# Autodesk Inventor assembly: Raspberry Pi 3
(part 2 of 2)
- C:\Users\jferner\Downloads\raspberry-pi-3-model-b-reference-design-solidworks-cad-rpi-raspberrypi-raspberry-pi-1.snapshot.83\Solidworks Complete Assembly\Raspberry Pi 3320.ipt
- C:\Users\jferner\Downloads\raspberry-pi-3-model-b-reference-design-solidworks-cad-rpi-raspberrypi-raspberry-pi-1.snapshot.83\Solidworks Complete Assembly\Raspberry Pi 3321.ipt
- C:\Users\jferner\Downloads\raspberry-pi-3-model-b-reference-design-solidworks-cad-rpi-raspberrypi-raspberry-pi-1.snapshot.83\Solidworks Complete Assembly\Raspberry Pi 3322.ipt
- C:\Users\jferner\Downloads\raspberry-pi-3-model-b-reference-design-solidworks-cad-rpi-raspberrypi-raspberry-pi-1.snapshot.83\Solidworks Complete Assembly\Raspberry Pi 3323.ipt
- C:\Users\jferner\Downloads\raspberry-pi-3-model-b-reference-design-solidworks-cad-rpi-raspberrypi-raspberry-pi-1.snapshot.83\Solidworks Complete Assembly\Raspberry Pi 3324.ipt
- C:\Users\jferner\Downloads\raspberry-pi-3-model-b-reference-design-solidworks-cad-rpi-raspberrypi-raspberry-pi-1.snapshot.83\Solidworks Complete Assembly\Raspberry Pi 3325.ipt
- C:\Users\jferner\Downloads\raspberry-pi-3-model-b-reference-design-solidworks-cad-rpi-raspberrypi-raspberry-pi-1.snapshot.83\Solidworks Complete Assembly\Raspberry Pi 3326.ipt
- C:\Users\jferner\Downloads\raspberry-pi-3-model-b-reference-design-solidworks-cad-rpi-raspberrypi-raspberry-pi-1.snapshot.83\Solidworks Complete Assembly\Raspberry Pi 3327.ipt
- C:\Users\jferner\Downloads\raspberry-pi-3-model-b-reference-design-solidworks-cad-rpi-raspberrypi-raspberry-pi-1.snapshot.83\Solidworks Complete Assembly\Raspberry Pi 3328.ipt
- C:\Users\jferner\Downloads\raspberry-pi-3-model-b-reference-design-solidworks-cad-rpi-raspberrypi-raspberry-pi-1.snapshot.83\Solidworks Complete Assembly\Raspberry Pi 3329.ipt
- C:\Users\jferner\Downloads\raspberry-pi-3-model-b-reference-design-solidworks-cad-rpi-raspberrypi-raspberry-pi-1.snapshot.83\Solidworks Complete Assembly\Raspberry Pi 3330.ipt
- C:\Users\jferner\Downloads\raspberry-pi-3-model-b-reference-design-solidworks-cad-rpi-raspberrypi-raspberry-pi-1.snapshot.83\Solidworks Complete Assembly\Raspberry Pi 3331.ipt
- C:\Users\jferner\Downloads\raspberry-pi-3-model-b-reference-design-solidworks-cad-rpi-raspberrypi-raspberry-pi-1.snapshot.83\Solidworks Complete Assembly\Raspberry Pi 3332.ipt
- C:\Users\jferner\Downloads\raspberry-pi-3-model-b-reference-design-solidworks-cad-rpi-raspberrypi-raspberry-pi-1.snapshot.83\Solidworks Complete Assembly\Raspberry Pi 3333.ipt
- C:\Users\jferner\Downloads\raspberry-pi-3-model-b-reference-design-solidworks-cad-rpi-raspberrypi-raspberry-pi-1.snapshot.83\Solidworks Complete Assembly\Raspberry Pi 3334.ipt
- C:\Users\jferner\Downloads\raspberry-pi-3-model-b-reference-design-solidworks-cad-rpi-raspberrypi-raspberry-pi-1.snapshot.83\Solidworks Complete Assembly\Raspberry Pi 3335.ipt
- C:\Users\jferner\Downloads\raspberry-pi-3-model-b-reference-design-solidworks-cad-rpi-raspberrypi-raspberry-pi-1.snapshot.83\Solidworks Complete Assembly\Raspberry Pi 3336.ipt
- C:\Users\jferner\Downloads\raspberry-pi-3-model-b-reference-design-solidworks-cad-rpi-raspberrypi-raspberry-pi-1.snapshot.83\Solidworks Complete Assembly\Raspberry Pi 3337.ipt
- C:\Users\jferner\Downloads\raspberry-pi-3-model-b-reference-design-solidworks-cad-rpi-raspberrypi-raspberry-pi-1.snapshot.83\Solidworks Complete Assembly\Raspberry Pi 3338.ipt
- C:\Users\jferner\Downloads\raspberry-pi-3-model-b-reference-design-solidworks-cad-rpi-raspberrypi-raspberry-pi-1.snapshot.83\Solidworks Complete Assembly\Raspberry Pi 3339.ipt
- C:\Users\jferner\Downloads\raspberry-pi-3-model-b-reference-design-solidworks-cad-rpi-raspberrypi-raspberry-pi-1.snapshot.83\Solidworks Complete Assembly\Raspberry Pi 3340.ipt
- C:\Users\jferner\Downloads\raspberry-pi-3-model-b-reference-design-solidworks-cad-rpi-raspberrypi-raspberry-pi-1.snapshot.83\Solidworks Complete Assembly\Raspberry Pi 3341.ipt
- C:\Users\jferner\Downloads\raspberry-pi-3-model-b-reference-design-solidworks-cad-rpi-raspberrypi-raspberry-pi-1.snapshot.83\Solidworks Complete Assembly\Raspberry Pi 3342.ipt
- C:\Users\jferner\Downloads\raspberry-pi-3-model-b-reference-design-solidworks-cad-rpi-raspberrypi-raspberry-pi-1.snapshot.83\Solidworks Complete Assembly\Raspberry Pi 3343.ipt
- C:\Users\jferner\Downloads\raspberry-pi-3-model-b-reference-design-solidworks-cad-rpi-raspberrypi-raspberry-pi-1.snapshot.83\Solidworks Complete Assembly\Raspberry Pi 3344.ipt
- C:\Users\jferner\Downloads\raspberry-pi-3-model-b-reference-design-solidworks-cad-rpi-raspberrypi-raspberry-pi-1.snapshot.83\Solidworks Complete Assembly\Raspberry Pi 3345.ipt
- C:\Users\jferner\Downloads\raspberry-pi-3-model-b-reference-design-solidworks-cad-rpi-raspberrypi-raspberry-pi-1.snapshot.83\Solidworks Complete Assembly\Raspberry Pi 3346.ipt
- C:\Users\jferner\Downloads\raspberry-pi-3-model-b-reference-design-solidworks-cad-rpi-raspberrypi-raspberry-pi-1.snapshot.83\Solidworks Complete Assembly\Raspberry Pi 3347.ipt
- C:\Users\jferner\Downloads\raspberry-pi-3-model-b-reference-design-solidworks-cad-rpi-raspberrypi-raspberry-pi-1.snapshot.83\Solidworks Complete Assembly\Raspberry Pi 3348.ipt
- C:\Users\jferner\Downloads\raspberry-pi-3-model-b-reference-design-solidworks-cad-rpi-raspberrypi-raspberry-pi-1.snapshot.83\Solidworks Complete Assembly\Raspberry Pi 3349.ipt
- C:\Users\jferner\Downloads\raspberry-pi-3-model-b-reference-design-solidworks-cad-rpi-raspberrypi-raspberry-pi-1.snapshot.83\Solidworks Complete Assembly\Raspberry Pi 3350.ipt
- C:\Users\jferner\Downloads\raspberry-pi-3-model-b-reference-design-solidworks-cad-rpi-raspberrypi-raspberry-pi-1.snapshot.83\Solidworks Complete Assembly\Raspberry Pi 3351.ipt
- C:\Users\jferner\Downloads\raspberry-pi-3-model-b-reference-design-solidworks-cad-rpi-raspberrypi-raspberry-pi-1.snapshot.83\Solidworks Complete Assembly\Raspberry Pi 3352.ipt
- C:\Users\jferner\Downloads\raspberry-pi-3-model-b-reference-design-solidworks-cad-rpi-raspberrypi-raspberry-pi-1.snapshot.83\Solidworks Complete Assembly\Raspberry Pi 3353.ipt
- C:\Users\jferner\Downloads\raspberry-pi-3-model-b-reference-design-solidworks-cad-rpi-raspberrypi-raspberry-pi-1.snapshot.83\Solidworks Complete Assembly\Raspberry Pi 3354.ipt
- C:\Users\jferner\Downloads\raspberry-pi-3-model-b-reference-design-solidworks-cad-rpi-raspberrypi-raspberry-pi-1.snapshot.83\Solidworks Complete Assembly\Raspberry Pi 3357.ipt
- C:\Users\jferner\Downloads\raspberry-pi-3-model-b-reference-design-solidworks-cad-rpi-raspberrypi-raspberry-pi-1.snapshot.83\Solidworks Complete Assembly\Raspberry Pi 3355.ipt
- C:\Users\jferner\Downloads\raspberry-pi-3-model-b-reference-design-solidworks-cad-rpi-raspberrypi-raspberry-pi-1.snapshot.83\Solidworks Complete Assembly\Raspberry Pi 3356.ipt
- C:\Users\jferner\Downloads\raspberry-pi-3-model-b-reference-design-solidworks-cad-rpi-raspberrypi-raspberry-pi-1.snapshot.83\Solidworks Complete Assembly\Part2^Raspberry Pi 3.ipt
- C:\Users\jferner\Downloads\raspberry-pi-3-model-b-reference-design-solidworks-cad-rpi-raspberrypi-raspberry-pi-1.snapshot.83\Solidworks Complete Assembly\Raspberry Pi 3360.ipt
- C:\Users\jferner\Downloads\raspberry-pi-3-model-b-reference-design-solidworks-cad-rpi-raspberrypi-raspberry-pi-1.snapshot.83\Solidworks Complete Assembly\Part4^Raspberry Pi 3.ipt
- C:\Users\jferner\Downloads\raspberry-pi-3-model-b-reference-design-solidworks-cad-rpi-raspberrypi-raspberry-pi-1.snapshot.83\Solidworks Complete Assembly\Solder2.ipt
- C:\Users\jferner\Downloads\raspberry-pi-3-model-b-reference-design-solidworks-cad-rpi-raspberrypi-raspberry-pi-1.snapshot.83\Solidworks Complete Assembly\Raspberry Pi 3358.ipt
- C:\Users\jferner\Downloads\raspberry-pi-3-model-b-reference-design-solidworks-cad-rpi-raspberrypi-raspberry-pi-1.snapshot.83\Solidworks Complete Assembly\Raspberry Pi 3359.ipt
- C:\Users\jferner\Downloads\raspberry-pi-3-model-b-reference-design-solidworks-cad-rpi-raspberrypi-raspberry-pi-1.snapshot.83\Solidworks Complete Assembly\mf-msmf050-2.ipt
- C:\Users\jferner\Downloads\raspberry-pi-3-model-b-reference-design-solidworks-cad-rpi-raspberrypi-raspberry-pi-1.snapshot.83\Solidworks Complete Assembly\Raspberry Pi 3163_smaller.ipt
- C:\Users\jferner\Downloads\raspberry-pi-3-model-b-reference-design-solidworks-cad-rpi-raspberrypi-raspberry-pi-1.snapshot.83\Solidworks Complete Assembly\Raspberry Pi 353_smaller.ipt
- C:\Users\jferner\Downloads\raspberry-pi-3-model-b-reference-design-solidworks-cad-rpi-raspberrypi-raspberry-pi-1.snapshot.83\Solidworks Complete Assembly\Raspberry Pi 3164_small.ipt
- C:\Users\jferner\Downloads\raspberry-pi-3-model-b-reference-design-solidworks-cad-rpi-raspberrypi-raspberry-pi-1.snapshot.83\Solidworks Complete Assembly\Raspberry Pi 3165_smaller.ipt
- C:\Users\jferner\Downloads\raspberry-pi-3-model-b-reference-design-solidworks-cad-rpi-raspberrypi-raspberry-pi-1.snapshot.83\Solidworks Complete Assembly\Raspberry Pi 3141_smaller.ipt
- C:\Users\jferner\Downloads\raspberry-pi-3-model-b-reference-design-solidworks-cad-rpi-raspberrypi-raspberry-pi-1.snapshot.83\Solidworks Complete Assembly\Assem1^Raspberry Pi 3.iam
- C:\Users\jferner\Downloads\raspberry-pi-3-model-b-reference-design-solidworks-cad-rpi-raspberrypi-raspberry-pi-1.snapshot.83\Solidworks Complete Assembly\raspberry_pi_B+_(microsd2).ipt
## Components (634 placed, 323 different names)
1. Raspberry Pi 3157:1
2. Raspberry Pi 3242:1
3. Raspberry Pi 3266:1
4. raspberry_pi_3(bar_180_2x20):2
5. RPi3_ModelB v1:1 [sub-assembly]
6. Raspberry Pi 312:1
7. Raspberry Pi 314:1
8. Raspberry Pi 3172:1
9. Raspberry Pi 3173:1
10. Raspberry Pi 3174:1
11. Raspberry Pi 3175:1
12. Raspberry Pi 3176:1
13. Raspberry Pi 3177:1
14. Raspberry Pi 3178:1
15. Raspberry Pi 3179:1
16. Raspberry Pi 3180:1
17. Raspberry Pi 3181:1
18. Raspberry Pi 3182:1
19. Raspberry Pi 3183:1
20. Raspberry Pi 3184:1
21. Raspberry Pi 3185:1
22. Raspberry Pi 3186:1
23. Raspberry Pi 3187:1
24. Raspberry Pi 3188:1
25. Raspberry Pi 3189:1
26. Raspberry Pi 3190:1
27. Raspberry Pi 3191:1
28. Raspberry Pi 3192:1
29. Raspberry Pi 3193:1
30. Raspberry Pi 3194:1
31. Raspberry Pi 3195:1
32. Raspberry Pi 3196:1
33. Raspberry Pi 3197:1
34. Raspberry Pi 3198:1
35. Raspberry Pi 3199:1
36. Raspberry Pi 3200:1
37. Raspberry Pi 3201:1
38. Raspberry Pi 3202:1
39. Raspberry Pi 3203:1
40. Raspberry Pi 3204:1
41. Raspberry Pi 3205:1
42. Raspberry Pi 3206:1
43. Raspberry Pi 3207:1
44. Raspberry Pi 3208:1
45. Raspberry Pi 3209:1
46. Raspberry Pi 3210:1
47. Raspberry Pi 3211:1
48. Raspberry Pi 3212:1
49. Raspberry Pi 3213:1
50. Raspberry Pi 3214:1
51. Raspberry Pi 3215:1
52. Raspberry Pi 3216:1
53. Raspberry Pi 3217:1
54. Raspberry Pi 3218:1
55. Raspberry Pi 3219:1
56. Raspberry Pi 3220:1
57. Raspberry Pi 3221:1
58. Raspberry Pi 3222:1
59. Raspberry Pi 3223:1
60. Raspberry Pi 3224:1
61. Raspberry Pi 3225:1
62. Raspberry Pi 3226:1
63. Raspberry Pi 3227:1
64. Raspberry Pi 3228:1
65. Raspberry Pi 3229:1
66. Raspberry Pi 3230:1
67. Raspberry Pi 3231:1
68. Raspberry Pi 3232:1
69. Raspberry Pi 3233:1
70. Raspberry Pi 3234:1
71. Raspberry Pi 3235:1
72. Raspberry Pi 31:1
73. Raspberry Pi 36:1
74. Raspberry Pi 32:1
75. Raspberry Pi 33:1
76. Raspberry Pi 34:1
77. Raspberry Pi 35:1
78. Raspberry Pi 37:1
79. Raspberry Pi 38:1
80. Raspberry Pi 39:1
81. Raspberry Pi 310:1
82. Raspberry Pi 311:1
83. Raspberry Pi 313:1
84. Raspberry Pi 315:1
85. Raspberry Pi 316:1
86. Raspberry Pi 317:1
87. Raspberry Pi 318:1
88. Raspberry Pi 319:1
89. Raspberry Pi 320:1
90. Raspberry Pi 322:1
91. Raspberry Pi 323:1
92. Raspberry Pi 324:1
93. Raspberry Pi 325:1
94. Raspberry Pi 326:1
95. Raspberry Pi 327:1
96. Raspberry Pi 328:1
97. Raspberry Pi 329:1
98. Raspberry Pi 330:1
99. Raspberry Pi 331:1
100. Raspberry Pi 332:1
101. Raspberry Pi 333:1
102. Raspberry Pi 334:1
103. Raspberry Pi 335:1
104. Raspberry Pi 336:1
105. Raspberry Pi 337:1
106. Raspberry Pi 338:1
107. Raspberry Pi 339:1
108. Raspberry Pi 340:1
109. Raspberry Pi 341:1
110. Raspberry Pi 342:1
111. Raspberry Pi 343:1
112. Raspberry Pi 344:1
113. Raspberry Pi 345:1
114. Raspberry Pi 346:1
115. Raspberry Pi 347:1
116. Raspberry Pi 348:1
117. Raspberry Pi 349:1
118. Raspberry Pi 350:1
119. Raspberry Pi 351:1
120. Raspberry Pi 352:1
121. Raspberry Pi 353:1
122. Raspberry Pi 354:1
123. Raspberry Pi 355:1
124. Raspberry Pi 356:1
125. Raspberry Pi 357:1
126. Raspberry Pi 358:1
127. Raspberry Pi 359:1
128. Raspberry Pi 360:1
129. Raspberry Pi 361:1
130. Raspberry Pi 362:1
131. Raspberry Pi 363:1
132. Raspberry Pi 364:1
133. Raspberry Pi 365:1
134. Raspberry Pi 366:1
135. Raspberry Pi 367:1
136. Raspberry Pi 368:1
137. Raspberry Pi 369:1
138. Raspberry Pi 370:1
139. Raspberry Pi 371:1
140. Raspberry Pi 372:1
141. Raspberry Pi 373:1
142. Raspberry Pi 374:1
143. Raspberry Pi 375:1
144. Raspberry Pi 376:1
145. Raspberry Pi 377:1
146. Raspberry Pi 378:1
147. Raspberry Pi 379:1
148. Raspberry Pi 380:1
149. Raspberry Pi 381:1
150. Raspberry Pi 382:1
151. Raspberry Pi 383:1
152. Raspberry Pi 385:1
153. Raspberry Pi 386:1
154. Raspberry Pi 387:1
155. Raspberry Pi 388:1
156. Raspberry Pi 390:1
157. Raspberry Pi 391:1
158. Raspberry Pi 393:1
159. Raspberry Pi 394:1
160. Raspberry Pi 395:1
161. Raspberry Pi 396:1
162. Raspberry Pi 397:1
163. Raspberry Pi 398:1
164. Raspberry Pi 399:1
165. Raspberry Pi 3100:1
166. Raspberry Pi 3101:1
167. Raspberry Pi 3102:1
168. Raspberry Pi 3103:1
169. Raspberry Pi 3104:1
170. Raspberry Pi 3105:1
171. Raspberry Pi 3106:1
172. Raspberry Pi 3107:1
173. Raspberry Pi 3108:1
174. Raspberry Pi 3109:1
175. Raspberry Pi 3110:1
176. Raspberry Pi 3111:1
177. Raspberry Pi 3112:1
178. Raspberry Pi 3113:1
179. Raspberry Pi 3114:1
180. Raspberry Pi 3115:1
181. Raspberry Pi 3116:1
182. Raspberry Pi 3117:1
183. Raspberry Pi 3118:1
184. Raspberry Pi 3119:1
185. Raspberry Pi 3120:1
186. Raspberry Pi 3121:1
187. Raspberry Pi 3122:1
188. Raspberry Pi 3123:1
189. Raspberry Pi 3124:1
190. Raspberry Pi 3125:1
191. Raspberry Pi 3126:1
192. Raspberry Pi 3127:1
193. Raspberry Pi 3128:1
194. Raspberry Pi 3129:1
195. Raspberry Pi 3130:1
196. Raspberry Pi 3131:1
197. Raspberry Pi 3132:1
198. Raspberry Pi 3133:1
199. Raspberry Pi 3134:1
200. Raspberry Pi 3135:1
201. Raspberry Pi 3137:1
202. Raspberry Pi 3138:1
203. Raspberry Pi 3139:1
204. Raspberry Pi 3140:1
205. Raspberry Pi 3141:1
206. Raspberry Pi 3142:1
207. Raspberry Pi 3143:1
208. Raspberry Pi 3144:1
209. Raspberry Pi 3146:1
210. Raspberry Pi 3147:1
211. Raspberry Pi 3149:1
212. Raspberry Pi 3150:1
213. Raspberry Pi 3151:1
214. Raspberry Pi 3152:1
215. Raspberry Pi 3153:1
216. Raspberry Pi 3154:1
217. Raspberry Pi 3155:1
218. Raspberry Pi 3156:1
219. Raspberry Pi 3158:1
220. Raspberry Pi 3159:1
221. Raspberry Pi 3160:1
222. Raspberry Pi 3161:1
223. Raspberry Pi 3162:1
224. Raspberry Pi 3163:1
225. Raspberry Pi 3164:1
226. Raspberry Pi 3165:1
227. Raspberry Pi 3166:1
228. Raspberry Pi 3167:1
229. Raspberry Pi 3168:1
230. Raspberry Pi 3169:1
231. Raspberry Pi 3170:1
232. Raspberry Pi 3171:1
233. Raspberry Pi 3276:1
234. Raspberry Pi 3277:1
235. Raspberry Pi 3278:1
236. Raspberry Pi 3279:1
237. Raspberry Pi 3280:1
238. Raspberry Pi 3281:1
239. Raspberry Pi 3282:1
240. Raspberry Pi 3283:1
241. Raspberry Pi 3284:1
242. Raspberry Pi 3285:1
243. Raspberry Pi 3286:1
244. Raspberry Pi 3287:1
245. Raspberry Pi 3288:1
246. Raspberry Pi 3289:1
247. Raspberry Pi 3290:1
248. Raspberry Pi 3291:1
249. Raspberry Pi 3292:1
250. Raspberry Pi 3293:1
251. Raspberry Pi 3294:1
252. Raspberry Pi 3295:1
253. Raspberry Pi 3296:1
254. Raspberry Pi 3297:1
255. Raspberry Pi 3298:1
256. Raspberry Pi 3299:1
257. Raspberry Pi 3300:1
258. Raspberry Pi 3301:1
259. Raspberry Pi 3302:1
260. Raspberry Pi 3303:1
261. Raspberry Pi 3304:1
262. Raspberry Pi 3305:1
263. Raspberry Pi 3306:1
264. Raspberry Pi 3307:1
265. Raspberry Pi 3308:1
266. Raspberry Pi 3309:1
267. Raspberry Pi 3310:1
268. Raspberry Pi 3311:1
269. Raspberry Pi 3312:1
270. Raspberry Pi 3313:1
271. Raspberry Pi 3314:1
272. Raspberry Pi 3315:1
273. Raspberry Pi 3316:1
274. Raspberry Pi 3317:1
275. Raspberry Pi 3318:1
276. Raspberry Pi 3319:1
277. Raspberry Pi 3320:1
278. Raspberry Pi 3321:1
279. Raspberry Pi 3322:1
280. Raspberry Pi 3323:1
281. Raspberry Pi 3324:1
282. Raspberry Pi 3325:1
283. Raspberry Pi 3326:1
284. Raspberry Pi 3327:1
285. Raspberry Pi 3328:1
286. Raspberry Pi 3329:1
287. Raspberry Pi 3330:1
288. Raspberry Pi 3331:1
289. Raspberry Pi 3332:1
290. Raspberry Pi 3333:1
291. Raspberry Pi 3334:1
292. Raspberry Pi 3335:1
293. Raspberry Pi 3336:1
294. Raspberry Pi 3337:1
295. Raspberry Pi 3338:1
296. Raspberry Pi 3339:1
297. Raspberry Pi 3340:1
298. Raspberry Pi 3341:1
299. Raspberry Pi 3342:1
300. Raspberry Pi 3343:1
301. Raspberry Pi 3344:1
302. Raspberry Pi 3345:1
303. Raspberry Pi 3346:1
304. Raspberry Pi 3347:1
305. Raspberry Pi 3348:1
306. Raspberry Pi 3349:1
307. Raspberry Pi 3350:1
308. Raspberry Pi 3351:1
309. Raspberry Pi 3352:1
310. Raspberry Pi 3353:1
311. Raspberry Pi 3354:1
312. Raspberry Pi 327:2
313. Raspberry Pi 340:2
314. Raspberry Pi 344:2
315. Raspberry Pi 344:3
316. Raspberry Pi 340:3
317. Raspberry Pi 344:4
318. Raspberry Pi 340:4
319. Raspberry Pi 344:6
320. Raspberry Pi 340:6
321. Raspberry Pi 344:7
322. Raspberry Pi 340:7
323. Raspberry Pi 340:8
324. Raspberry Pi 344:8
325. Raspberry Pi 340:9
326. Raspberry Pi 344:9
327. Raspberry Pi 3357:1
328. Raspberry Pi 3355:1
329. Raspberry Pi 3356:1
330. Raspberry Pi 374:2
331. Raspberry Pi 3141:2
332. Raspberry Pi 374:3
333. Raspberry Pi 374:4
334. Raspberry Pi 374:5
335. Part2^Raspberry Pi 3:1
336. Raspberry Pi 3360:1
337. Part4^Raspberry Pi 3:1
338. Raspberry Pi 3159:2
339. Raspberry Pi 3158:2
340. Raspberry Pi 3160:2
341. Raspberry Pi 3162:2
342. Raspberry Pi 3161:2
343. Raspberry Pi 359:2
344. Raspberry Pi 3165:2
345. Raspberry Pi 353:2
346. Raspberry Pi 3164:2
347. Raspberry Pi 3163:2
348. Raspberry Pi 355:3
349. Raspberry Pi 3168:3
350. Raspberry Pi 3170:3
351. Raspberry Pi 3169:3
352. Raspberry Pi 3171:3
353. Raspberry Pi 3167:3
354. Raspberry Pi 3166:3
355. Raspberry Pi 353:3
356. Raspberry Pi 3165:3
357. Raspberry Pi 3163:3
358. Raspberry Pi 3164:3
359. Solder2:1
360. Solder2:41
361. Solder2:42
362. Solder2:43
363. Solder2:44
364. Solder2:45
365. Solder2:46
366. Solder2:47
367. Solder2:48
368. Solder2:49
369. Solder2:59
370. Raspberry Pi 3358:1
371. Raspberry Pi 3359:1
372. Solder2:68
373. Solder2:69
374. Solder2:70
375. Solder2:71
376. Solder2:72
377. Solder2:73
378. Solder2:74
379. Solder2:75
380. Solder2:76
381. Solder2:77
382. Solder2:78
383. Solder2:79
384. mf-msmf050-2:1
385. Solder2:87
386. Raspberry Pi 3163:4
387. Raspberry Pi 353:4
388. Raspberry Pi 3164:4
389. Raspberry Pi 3165:4
390. Raspberry Pi 3163:5
391. Raspberry Pi 353:5
392. Raspberry Pi 3164:5
393. Raspberry Pi 3165:5
394. Raspberry Pi 3163:6
395. Raspberry Pi 353:6
396. Raspberry Pi 3164:6
397. Raspberry Pi 3165:6
398. Raspberry Pi 3141:3
399. Raspberry Pi 3141:4
400. Raspberry Pi 3141:5
401. Raspberry Pi 3141:6
402. Raspberry Pi 3141:7
403. Raspberry Pi 3141:8
404. Raspberry Pi 3141:9
405. Raspberry Pi 3141:10
406. Raspberry Pi 3141:11
407. Raspberry Pi 3141:12
408. Raspberry Pi 3141:13
409. Raspberry Pi 3141:14
410. Raspberry Pi 3141:15
411. Raspberry Pi 3141:17
412. Raspberry Pi 3141:18
413. Raspberry Pi 3141:19
414. Raspberry Pi 3141:20
415. Raspberry Pi 3141:21
416. Raspberry Pi 3141:22
417. Raspberry Pi 3141:23
418. Raspberry Pi 3141:24
419. Raspberry Pi 3141:25
420. Raspberry Pi 3141:26
421. Raspberry Pi 3141:27
422. Raspberry Pi 3141:28
423. Raspberry Pi 3141:29
424. Raspberry Pi 3141:30
425. Raspberry Pi 3141:31
426. Raspberry Pi 3141:32
427. Raspberry Pi 3141:35
428. Raspberry Pi 3141:36
429. Raspberry Pi 3141:37
430. Raspberry Pi 3141:38
431. Raspberry Pi 3141:39
432. Raspberry Pi 3141:40
433. Raspberry Pi 3141:41
434. Raspberry Pi 3141:42
435. Raspberry Pi 3141:43
436. Raspberry Pi 3141:44
437. Raspberry Pi 3141:45
438. Raspberry Pi 3141:46
439. Raspberry Pi 3141:47
440. Raspberry Pi 3141:48
441. Raspberry Pi 3141:49
442. Raspberry Pi 3141:50
443. Raspberry Pi 3141:51
444. Raspberry Pi 3141:52
445. Raspberry Pi 3141:53
446. Raspberry Pi 3141:54
447. Raspberry Pi 3141:55
448. Raspberry Pi 3141:56
449. Raspberry Pi 3141:57
450. Raspberry Pi 3141:58
451. Raspberry Pi 3141:59
452. Raspberry Pi 3141:60
453. Raspberry Pi 3141:61
454. Raspberry Pi 3141:62
455. Raspberry Pi 3141:63
456. Raspberry Pi 374:6
457. Raspberry Pi 3141:66
458. Raspberry Pi 3141:67
459. Raspberry Pi 3141:68
460. Raspberry Pi 3141:69
461. Raspberry Pi 3141:70
462. Raspberry Pi 3141:72
463. Raspberry Pi 3141:73
464. Raspberry Pi 3141:74
465. Raspberry Pi 3141:75
466. Raspberry Pi 3141:76
467. Raspberry Pi 3141:77
468. Raspberry Pi 3141:78
469. Raspberry Pi 3141:79
470. Raspberry Pi 3141:80
471. Raspberry Pi 3141:82
472. Raspberry Pi 3141:84
473. Raspberry Pi 3141:86
474. Raspberry Pi 3141:88
475. Raspberry Pi 3141:89
476. Raspberry Pi 3141:90
477. Raspberry Pi 3141:91
478. Raspberry Pi 3141:92
479. Raspberry Pi 3141:93
480. Raspberry Pi 3141:95
481. Raspberry Pi 3141:96
482. Raspberry Pi 3141:97
483. Raspberry Pi 3141:98
484. Raspberry Pi 3141:100
485. Raspberry Pi 3141:101
486. Raspberry Pi 3141:102
487. Raspberry Pi 3141:103
488. Raspberry Pi 3141:104
489. Raspberry Pi 3141:105
490. Raspberry Pi 3141:106
491. Raspberry Pi 3141:107
492. Raspberry Pi 3141:108
493. Raspberry Pi 3141:109
494. Raspberry Pi 3141:110
495. Raspberry Pi 3141:112
496. Raspberry Pi 3141:113
497. Raspberry Pi 3141:114
498. Raspberry Pi 3141:115
499. Raspberry Pi 3141:116
500. Raspberry Pi 3141:117
501. Raspberry Pi 3141:118
502. Raspberry Pi 3141:119
503. Raspberry Pi 3141:120
504. Raspberry Pi 3141:121
505. Raspberry Pi 3141:122
506. Raspberry Pi 3141:123
507. Raspberry Pi 3141:124
508. Raspberry Pi 3141:126
509. Raspberry Pi 3281:2
510. Raspberry Pi 3280:2
511. Raspberry Pi 3282:2
512. Raspberry Pi 3285:2
513. Raspberry Pi 3283:2
514. Raspberry Pi 3284:2
515. Raspberry Pi 34:2
516. Raspberry Pi 3141:128
517. Raspberry Pi 3141:129
518. Raspberry Pi 3141:130
519. Raspberry Pi 3141:131
520. Raspberry Pi 3141:132
521. Raspberry Pi 3141:133
522. Raspberry Pi 3141:134
523. Raspberry Pi 3141:135
524. Raspberry Pi 3141:137
525. Raspberry Pi 3141:138
526. Raspberry Pi 3141:139
527. Raspberry Pi 3141:140
528. Raspberry Pi 3141:141
529. Raspberry Pi 3141:143
530. Raspberry Pi 3141:145
531. Raspberry Pi 345:2
532. Raspberry Pi 345:3
533. Raspberry Pi 345:4
534. Raspberry Pi 345:5
535. Assem1^Raspberry Pi 3:1 [sub-assembly]
536. Raspberry Pi 3141:147
537. Solder2:2
538. Solder2:3
539. Solder2:4
540. Solder2:5
541. Solder2:6
542. Solder2:7
543. Solder2:8
544. Solder2:9
545. Solder2:10
546. Solder2:11
547. Solder2:12
548. Solder2:13
549. Solder2:14
550. Solder2:15
551. Solder2:16
552. Solder2:17
553. Solder2:18
554. Solder2:19
555. Solder2:20
556. Solder2:21
557. Solder2:22
558. Solder2:23
559. Solder2:24
560. Solder2:25
561. Solder2:26
562. Solder2:27
563. Solder2:28
564. Solder2:29
565. Solder2:30
566. Solder2:31
567. Solder2:32
568. Solder2:33
569. Solder2:34
570. Solder2:35
571. Solder2:36
572. Solder2:37
573. Solder2:38
574. Solder2:39
575. Solder2:40
576. Solder2:51
577. Solder2:52
578. Solder2:53
579. Solder2:54
580. Solder2:55
581. Solder2:56
582. Solder2:57
583. Solder2:61
584. Solder2:62
585. Solder2:63
586. Solder2:64
587. Solder2:65
588. Solder2:66
589. Solder2:67
590. Solder2:81
591. Solder2:82
592. Solder2:83
593. Solder2:84
594. Solder2:85
595. Solder2:86
596. raspberry_pi_B+_(microsd2):1
597. Raspberry Pi 3242:2
598. Raspberry Pi 3242:3
599. Raspberry Pi 3242:4
600. Raspberry Pi 3242:5
601. Raspberry Pi 3242:6
602. Raspberry Pi 3242:7
603. Raspberry Pi 3242:8
604. Raspberry Pi 3242:9
605. Raspberry Pi 3242:10
606. Raspberry Pi 3242:11
607. Raspberry Pi 3242:12
608. Raspberry Pi 3242:13
609. Raspberry Pi 3242:14
610. Raspberry Pi 3242:15
611. Raspberry Pi 3242:16
612. Raspberry Pi 3242:17
613. Raspberry Pi 3242:18
614. Raspberry Pi 3242:19
615. Raspberry Pi 3242:20
616. Raspberry Pi 3266:2
617. Raspberry Pi 3266:3
618. Raspberry Pi 3266:4
619. Raspberry Pi 3266:5
620. Raspberry Pi 3266:6
621. Raspberry Pi 3266:7
622. Raspberry Pi 3266:8
623. Raspberry Pi 3266:9
624. Raspberry Pi 3266:10
625. Raspberry Pi 3266:11
626. Raspberry Pi 3266:12
627. Raspberry Pi 3266:13
628. Raspberry Pi 3266:14
629. Raspberry Pi 3266:15
630. Raspberry Pi 3266:16
631. Raspberry Pi 3266:17
632. Raspberry Pi 3266:18
633. Raspberry Pi 3266:19
634. Raspberry Pi 3266:20
